# Autodesk Inventor assembly: BLTouch-WiringSocket - Assembly
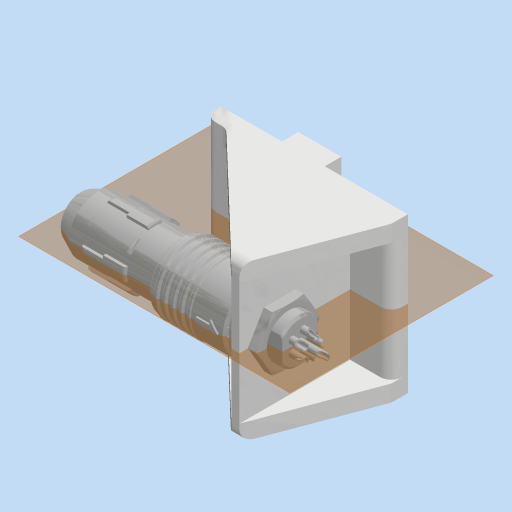
[picture p0: Inventor's stored thumbnail of the model, 512x512]
Saved by Autodesk Inventor 2023.2 (Build 272271000, 271)
## iProperties
Created: 2024-02-16
Part Number: BLTouch-WiringSocket - Assembly
Document SubType Name: Assembly
Designer: Nils Bade
Author: Nils Bade
## Documents named in this file (6)
- C:\Users\nilsb\Documents\Inventor\Projektarbeit-Bade\RatRig_modified\ProbeHead\BLTouch-WiringSocket - Assembly.iam
- C:\Users\nilsb\Documents\Inventor\Projektarbeit-Bade\RatRig_modified\ProbeHead\BLTouch-WiringSocket.ipt
- C:\Users\nilsb\Documents\Inventor\Projektarbeit-Bade\RatRig_modified\T-NUT - DropIn 4040 SERIES - M6.ipt
- C:\Users\nilsb\Documents\Inventor\Projektarbeit-Bade\Schrauben\Cap Head Screw M6x12 v2.ipt
- C:\Users\nilsb\Documents\Inventor\Projektarbeit-Bade\RatRig_modified\ProbeHead\HR30-6R-6S - Jack.ipt
- C:\Users\nilsb\Documents\Inventor\Projektarbeit-Bade\RatRig_modified\ProbeHead\HR30-6PA-6P - Plug.ipt
## Components (5 placed, 5 different names)
1. BLTouch-WiringSocket:1 — Passend:1, Winkel:1, Passend:2, Passend:3, Passend:4, Winkel:2, Passend:5, Passend:6
2. T-NUT - DROP IN TYPE FOR 40 SERIES - M6:1 — Passend:1, Winkel:1, Passend:2
3. Cap Head Screw M6x12 v2:1 — Passend:3, Passend:4
4. HR30-6R-6S - Jack:1 — Winkel:2, Passend:5, Passend:6, Passend:7, Winkel:3, Passend:8
5. HR30-6PA-6P - Plug:1 — Passend:7, Winkel:3, Passend:8
## Relationships (11: Mate 8, Angle 3)
- Passend:1 [Mate]: BLTouch-WiringSocket:1 ↔ T-NUT - DROP IN TYPE FOR 40 SERIES - M6:1
- Winkel:1 [Angle] (0 deg): BLTouch-WiringSocket:1 ↔ T-NUT - DROP IN TYPE FOR 40 SERIES - M6:1
- Passend:2 [Mate] (4.5 mm): BLTouch-WiringSocket:1 ↔ T-NUT - DROP IN TYPE FOR 40 SERIES - M6:1
- Passend:3 [Mate]: BLTouch-WiringSocket:1 ↔ Cap Head Screw M6x12 v2:1
- Passend:4 [Mate]: BLTouch-WiringSocket:1 ↔ Cap Head Screw M6x12 v2:1
- Winkel:2 [Angle] (0 deg): BLTouch-WiringSocket:1 ↔ HR30-6R-6S - Jack:1
- Passend:5 [Mate]: BLTouch-WiringSocket:1 ↔ HR30-6R-6S - Jack:1
- Passend:6 [Mate]: BLTouch-WiringSocket:1 ↔ HR30-6R-6S - Jack:1
- Passend:7 [Mate]: HR30-6R-6S - Jack:1 ↔ HR30-6PA-6P - Plug:1
- Winkel:3 [Angle] (180 deg): HR30-6R-6S - Jack:1 ↔ HR30-6PA-6P - Plug:1
- Passend:8 [Mate]: HR30-6R-6S - Jack:1 ↔ HR30-6PA-6P - Plug:1
